# Autodesk Inventor assembly: Full_HITscope_v1
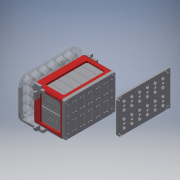
[picture p0: Inventor's stored thumbnail of the model, 180x180]
Saved by Autodesk Inventor 2019.4 (Build 234330000, 330)
## iProperties
Created: 2021-09-09
Part Number: Full_HITscope_v1
Material: Generisch
Document SubType Name: Assembly
Designer: Muriel
Mass: 256.869 g
Surface Area: 2541.25 cm^2
Volume: 256.869 cm^3
Density: 1 g/cm^3
Author: Muriel
## Documents named in this file (10)
- C:\Users\diederichbenedict\Dropbox\Dokumente\Promotion\PROJECTS\Omniscope\INVENTOR\Full_HITscope_v1.iam
- C:\Users\diederichbenedict\Dropbox\Dokumente\Promotion\PROJECTS\Omniscope\INVENTOR\Assembly_Omniscope_v1.iam
- C:\Users\diederichbenedict\Dropbox\Dokumente\Promotion\PROJECTS\Omniscope\INVENTOR\05_Omniscope_base_v1.ipt
- C:\Users\diederichbenedict\Dropbox\Dokumente\Promotion\PROJECTS\Omniscope\INVENTOR\06_Omniscope_lid_lenses.ipt
- C:\Users\diederichbenedict\Dropbox\Dokumente\Promotion\PROJECTS\Omniscope\INVENTOR\07_Omnivision_Lamp_arm.ipt
- C:\Users\diederichbenedict\Dropbox\Dokumente\Promotion\PROJECTS\Omniscope\INVENTOR\02_Omniscope_lid_bottom.ipt
- C:\Users\diederichbenedict\Dropbox\Dokumente\Promotion\PROJECTS\UC2\02_CAD\INVENTOR\uc2_v3\00_24wellplate_base_2.ipt
- C:\Users\diederichbenedict\Dropbox\Dokumente\Promotion\PROJECTS\Omniscope\INVENTOR\03_Omniscope_lid_lenses.ipt
- C:\Users\diederichbenedict\Dropbox\Dokumente\Promotion\PROJECTS\Omniscope\INVENTOR\07_Omnivision_wellplate_traystage.ipt
- C:\Users\diederichbenedict\Dropbox\Dokumente\Promotion\PROJECTS\Omniscope\INVENTOR\00_Microlinearmotor.ipt
## Components (23 placed, 9 different names)
1. 05_Omniscope_base_v1:1 — Fluchtend:5, Fluchtend:6, Einfügen:2, Flush:7, Angle:2, Flush:8, Mate:1, Flush:9, Flush:10, Mate:3, Flush:13, Mate:4, Mate:5, Flush:14, Mate:7, Flush:15
2. 07_Omnivision_Lamp_arm:1 — Fluchtend:5, Fluchtend:6
3. 07_Omnivision_Lamp_arm:2 — Einfügen:2
4. 02_Omniscope_lid_bottom:1 — Flush:7, Insert:3
5. 06_Omniscope_lid_lenses:1
6. 00_24wellplate_base_2:1 — Flush:8, Mate:1, Flush:11, Flush:12
7. 03_Omniscope_lid_lenses:1 — Flush:9, Flush:10, Mate:6
8. 07_Omnivision_wellplate_traystage:1 — Flush:11, Flush:12
9. 00_Microlinearmotor:1 — Mate:3, Flush:13, Mate:4, Flush:16
10. 00_Microlinearmotor:2 — Mate:5, Flush:14, Mate:6
11. 00_Microlinearmotor:3 — Mate:7, Flush:15, Flush:16
12. Assembly_Omniscope_v1:1 [sub-assembly] — Insert:3, Angle:2
13. Assembly_Omniscope_v1:2 [sub-assembly]
14. Assembly_Omniscope_v1:3 [sub-assembly]
15. Assembly_Omniscope_v1:4 [sub-assembly]
16. Assembly_Omniscope_v1:5 [sub-assembly]
17. Assembly_Omniscope_v1:6 [sub-assembly]
18. Assembly_Omniscope_v1:7 [sub-assembly]
19. Assembly_Omniscope_v1:8 [sub-assembly]
20. Assembly_Omniscope_v1:9 [sub-assembly]
21. Assembly_Omniscope_v1:10 [sub-assembly]
22. Assembly_Omniscope_v1:11 [sub-assembly]
23. Assembly_Omniscope_v1:12 [sub-assembly]
## Component patterns: (12 elements, first: Assembly_Omniscope_v1:1)
## Relationships (21: Flush 12, Mate 6, Insert 2, Angle 1)
- Fluchtend:5 [Flush]: 05_Omniscope_base_v1:1 ↔ 07_Omnivision_Lamp_arm:1
- Fluchtend:6 [Flush]: 05_Omniscope_base_v1:1 ↔ 07_Omnivision_Lamp_arm:1
- Einfügen:2 [Insert]: 05_Omniscope_base_v1:1 ↔ 07_Omnivision_Lamp_arm:2
- Flush:7: 05_Omniscope_base_v1:1 ↔ 02_Omniscope_lid_bottom:1
- Insert:3: 02_Omniscope_lid_bottom:1 ↔ Assembly_Omniscope_v1:1
- Angle:2 (0 deg): 05_Omniscope_base_v1:1 ↔ Assembly_Omniscope_v1:1
- Flush:8: 05_Omniscope_base_v1:1 ↔ 00_24wellplate_base_2:1
- Mate:1 (2 mm): 05_Omniscope_base_v1:1 ↔ 00_24wellplate_base_2:1
- Flush:9: 05_Omniscope_base_v1:1 ↔ 03_Omniscope_lid_lenses:1
- Flush:10: 05_Omniscope_base_v1:1 ↔ 03_Omniscope_lid_lenses:1
- Flush:11: 00_24wellplate_base_2:1 ↔ 07_Omnivision_wellplate_traystage:1
- Flush:12: 00_24wellplate_base_2:1 ↔ 07_Omnivision_wellplate_traystage:1
- Mate:3: 05_Omniscope_base_v1:1 ↔ 00_Microlinearmotor:1
- Flush:13 (1 mm): 05_Omniscope_base_v1:1 ↔ 00_Microlinearmotor:1
- Mate:4 (1 mm): 05_Omniscope_base_v1:1 ↔ 00_Microlinearmotor:1
- Mate:5: 05_Omniscope_base_v1:1 ↔ 00_Microlinearmotor:2
- Flush:14 (1 mm): 05_Omniscope_base_v1:1 ↔ 00_Microlinearmotor:2
- Mate:6 (1 mm): 03_Omniscope_lid_lenses:1 ↔ 00_Microlinearmotor:2
- Mate:7: 05_Omniscope_base_v1:1 ↔ 00_Microlinearmotor:3
- Flush:15 (1 mm): 05_Omniscope_base_v1:1 ↔ 00_Microlinearmotor:3
- Flush:16: 00_Microlinearmotor:1 ↔ 00_Microlinearmotor:3
